# Autodesk Inventor assembly: Swerve-Drivetrain-2
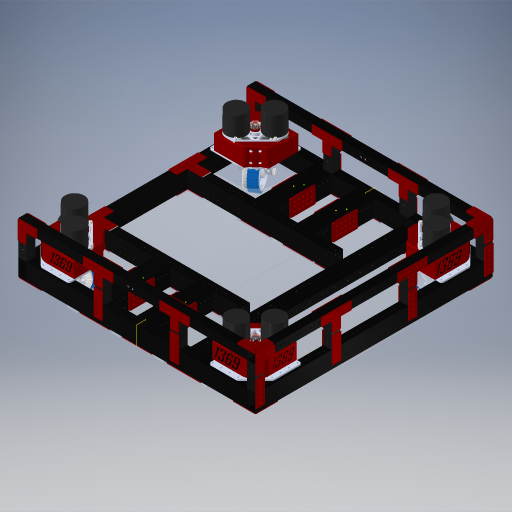
[picture p0: Inventor's stored thumbnail of the model, 512x512]
Saved by Autodesk Inventor 2024.2 (Build 282272000, 272)
## iProperties
Created: 2024-01-06
Part Number: Swerve-Drivetrain-2
Document SubType Name: Assembly
Designer: rohan
Author: rohan
## Documents named in this file (18)
- C:\Users\rohan\OneDrive - Hillsborough County Public Schools\Robotics\FIRST-Robotics-Competition\Crescendo\Minotaur-Crescendo-Robot\Swerve-Drivetrain.iam
- C:\Users\rohan\OneDrive - Hillsborough County Public Schools\Robotics\FIRST-Robotics-Competition\Crescendo\Minotaur-Crescendo-Robot\Motion\SDS-Swerve-Modules\MK3-Swerve-Module-Neos.iam
- C:\Users\rohan\OneDrive - Hillsborough County Public Schools\Robotics\FIRST-Robotics-Competition\Crescendo\Minotaur-Crescendo-Robot\Structure\Aluminum-Extrusions\2024-100-002-Front-Back-Extrusions.ipt
- C:\Users\rohan\OneDrive - Hillsborough County Public Schools\Robotics\FIRST-Robotics-Competition\Crescendo\Minotaur-Crescendo-Robot\Structure\Aluminum-Extrusions\2024-100-001-Left-Right-Extrusions.ipt
- C:\Users\rohan\OneDrive - Hillsborough County Public Schools\Robotics\FIRST-Robotics-Competition\Crescendo\Minotaur-Crescendo-Robot\Structure\Aluminum-Extrusions\2024-100-003-Middle-Extrusions.ipt
- C:\Users\rohan\OneDrive - Hillsborough County Public Schools\Robotics\FIRST-Robotics-Competition\Crescendo\Minotaur-Crescendo-Robot\Structure\Gussets\THRIFYBOT-L-Gusset.ipt
- C:\Users\rohan\OneDrive - Hillsborough County Public Schools\Robotics\FIRST-Robotics-Competition\Crescendo\Minotaur-Crescendo-Robot\Structure\Bumpers.ipt
- C:\Users\rohan\OneDrive - Hillsborough County Public Schools\Robotics\FIRST-Robotics-Competition\Crescendo\Minotaur-Crescendo-Robot\Structure\Aluminum-Extrusions\2024-100-007-Front-B-Tubing-Mount.ipt
- C:\Users\rohan\OneDrive - Hillsborough County Public Schools\Robotics\FIRST-Robotics-Competition\Crescendo\Minotaur-Crescendo-Robot\Structure\Gussets\THRIFYBOT-T-Gusset.ipt
- C:\Users\rohan\OneDrive - Hillsborough County Public Schools\Robotics\FIRST-Robotics-Competition\Crescendo\Minotaur-Crescendo-Robot\Structure\Gussets\Custom-Underside-T-Gusset.ipt
- C:\Users\rohan\OneDrive - Hillsborough County Public Schools\Robotics\FIRST-Robotics-Competition\Crescendo\Minotaur-Crescendo-Robot\Structure\Gussets\Custom-Underside-L-Gusset.ipt
- C:\Users\rohan\OneDrive - Hillsborough County Public Schools\Robotics\FIRST-Robotics-Competition\Crescendo\Minotaur-Crescendo-Robot\Structure\Aluminum-Extrusions\Superstructure-Mount.iam
- C:\Users\rohan\OneDrive - Hillsborough County Public Schools\Robotics\FIRST-Robotics-Competition\Crescendo\Minotaur-Crescendo-Robot\Structure\Gussets\3x5-Grid-Gusset.ipt
- C:\Users\rohan\OneDrive - Hillsborough County Public Schools\Robotics\FIRST-Robotics-Competition\Crescendo\Minotaur-Crescendo-Robot\Structure\Aluminum-Extrusions\2024-100-005-Climber-Mount.ipt
- C:\Users\rohan\OneDrive - Hillsborough County Public Schools\Robotics\FIRST-Robotics-Competition\Crescendo\Minotaur-Crescendo-Robot\Structure\Aluminum-Extrusions\2024-100-010-Climber-Support.ipt
- C:\Users\rohan\OneDrive - Hillsborough County Public Schools\Robotics\FIRST-Robotics-Competition\Crescendo\Minotaur-Crescendo-Robot\Structure\Gussets\1x5-Grid-Gusset.ipt
- C:\Users\rohan\OneDrive - Hillsborough County Public Schools\Robotics\FIRST-Robotics-Competition\Crescendo\Minotaur-Crescendo-Robot\Structure\Aluminum-Plates\2024-100-006-Electrical-Plate-Bottom.ipt
- C:\Users\rohan\OneDrive - Hillsborough County Public Schools\Robotics\FIRST-Robotics-Competition\Crescendo\Minotaur-Crescendo-Robot\Structure\Aluminum-Plates\2024-100-006-Electrical-Plate-Front.ipt
## Components (61 placed, 17 different names)
1. MK3-Swerve-Module-Neos:1 [sub-assembly] — Mate:75, Mate:80, Mate:81
2. MK3-Swerve-Module-Neos:2 [sub-assembly] — Mate:74, Mate:82, Mate:83
3. MK3-Swerve-Module-Neos:3 [sub-assembly] — Mate:73, Mate:76, Mate:77
4. MK3-Swerve-Module-Neos:4 [sub-assembly] — Mate:72, Mate:78, Mate:79
5. 2024-100-001-Left-Right-Extrusions:1 — Mate:69, Flush:1, Flush:2, Mate:70, Flush:3, Flush:4, Mate:73, Mate:76, Mate:82, Flush:12, Flush:14, Flush:45, Mate:111, Flush:53, Flush:54, Mate:147, Mate:148, Mate:149, Flush:106, Flush:107, Insert:14, Insert:15, Mate:165, Mate:166
6. 2024-100-001-Left-Right-Extrusions:2 — Mate:71, Flush:5, Flush:6, Mate:79, Mate:81, Flush:10, Flush:16, Mate:99, Mate:106, Flush:51, Flush:88, Flush:91, Mate:157, Mate:158, Flush:109, Flush:111
7. 2024-100-002-Front-Back-Extrusions:1 — Mate:70, Flush:3, Flush:4, Mate:72, Mate:77, Mate:78, Mate:88, Mate:89, Flush:13, Flush:15, Flush:33, Mate:112, Mate:159, Mate:160, Mate:161, Mate:162, Mate:163, Mate:164, Flush:110
8. 2024-100-002-Front-Back-Extrusions:2 — Mate:69, Flush:1, Flush:2, Mate:71, Flush:5, Flush:6, Mate:74, Mate:75, Mate:80, Mate:83, Mate:86, Mate:87, Flush:9, Flush:11, Mate:98, Mate:101, Flush:38, Flush:40, Insert:1, Flush:43, Mate:105, Insert:2, Flush:55, Mate:123, Mate:167, Flush:108
9. THRIFYBOT-L-Gusset:1 — Mate:89, Flush:13, Flush:14
10. THRIFYBOT-L-Gusset:2 — Mate:88, Flush:15, Flush:16
11. THRIFYBOT-L-Gusset:3 — Mate:87, Flush:11, Flush:12
12. THRIFYBOT-L-Gusset:4 — Mate:86, Flush:9, Flush:10
13. Bumpers:1 — Mate:98, Mate:99, Flush:33
14. 2024-100-007-Front-B-Tubing-Mount:1 — Mate:100, Flush:34, Mate:101, Flush:35, Flush:39, Mate:103, Flush:40, Mate:107, Flush:48, Insert:3, Mate:121, Flush:70, Mate:136, Flush:87, Flush:89, Mate:140, Flush:90, Insert:20
15. 2024-100-007-Front-B-Tubing-Mount:2 — Mate:100, Flush:34, Flush:35, Flush:44, Flush:47, Insert:4, Flush:102, Flush:103, Flush:104, Flush:105, Insert:16, Insert:17
16. THRIFYBOT-T-Gusset:1 — Flush:36, Mate:102, Flush:37, Mate:103
17. THRIFYBOT-T-Gusset:2 — Flush:36, Mate:102, Flush:37, Flush:38, Flush:39, Insert:1
18. THRIFYBOT-T-Gusset:3 — Mate:105
19. THRIFYBOT-T-Gusset:4 — Flush:43, Flush:44, Insert:2
20. 2024-100-003-Middle-Extrusions:1 — Flush:45, Mate:106, Mate:107, Mate:108, Mate:109, Flush:46, Flush:49, Mate:110, Flush:50, Flush:52, Mate:168
21. Custom-Underside-T-Gusset:1 — Mate:108, Flush:48, Flush:49, Insert:3
22. Custom-Underside-T-Gusset:2 — Mate:109, Flush:46, Flush:47, Insert:4
23. Custom-Underside-L-Gusset:4 — Mate:111, Flush:52, Flush:53
24. Custom-Underside-L-Gusset:5 — Mate:110, Flush:50, Flush:51
25. Superstructure-Mount:1 [sub-assembly] — Mate:112, Flush:54, Flush:55, Insert:21, Insert:22, Insert:23, Insert:24, Insert:25, Insert:26, Insert:27, Insert:28, Insert:29, Insert:30, Insert:31, Insert:32, Insert:33, Insert:34, Insert:35, Insert:36, Insert:37, Insert:38, Insert:39, Insert:40
26. 3x5-Grid-Gusset:3
27. 3x5-Grid-Gusset:4
28. 2024-100-005-Climber-Mount:2 — Flush:70, Mate:123
29. 2024-100-010-Climber-Support:2 — Mate:121, Mate:137, Mate:138, Insert:10, Insert:11
30. 3x5-Grid-Gusset:5
31. 3x5-Grid-Gusset:6
32. 2024-100-005-Climber-Mount:3 — Mate:136, Flush:87
33. 2024-100-010-Climber-Support:3 — Mate:139, Insert:8, Insert:9
34. THRIFYBOT-T-Gusset:5 — Mate:139, Flush:91, Insert:8
35. THRIFYBOT-T-Gusset:6 — Flush:89, Mate:138, Insert:11
36. THRIFYBOT-T-Gusset:7 — Mate:140, Flush:90, Insert:9, Insert:20
37. THRIFYBOT-T-Gusset:8 — Mate:137, Flush:88, Insert:10
38. 3x5-Grid-Gusset:7
39. 3x5-Grid-Gusset:8
40. 2024-100-005-Climber-Mount:4 — Mate:147, Flush:103
41. 2024-100-010-Climber-Support:4 — Mate:150, Mate:152, Insert:18
42. 3x5-Grid-Gusset:9
43. 3x5-Grid-Gusset:10
44. 2024-100-005-Climber-Mount:5 — Flush:102
45. 2024-100-010-Climber-Support:5 — Mate:148, Mate:151, Insert:19
46. THRIFYBOT-T-Gusset:9 — Mate:149, Flush:106, Insert:15, Insert:19
47. THRIFYBOT-T-Gusset:10 — Mate:151, Flush:105, Insert:16
48. THRIFYBOT-T-Gusset:11 — Mate:150, Flush:107, Insert:14, Insert:18
49. THRIFYBOT-T-Gusset:12 — Mate:152, Flush:104, Insert:17
50. 1x5-Grid-Gusset:1 — Mate:157, Insert:21, Insert:22
51. 1x5-Grid-Gusset:2 — Mate:158, Insert:23, Insert:24
52. 1x5-Grid-Gusset:3 — Mate:159, Insert:27, Insert:28
53. 1x5-Grid-Gusset:4 — Mate:160, Insert:25, Insert:26
54. 1x5-Grid-Gusset:5 — Mate:161, Insert:31, Insert:32
55. 1x5-Grid-Gusset:6 — Mate:162, Insert:29, Insert:30
56. 1x5-Grid-Gusset:7 — Mate:163, Insert:33, Insert:34
57. 1x5-Grid-Gusset:8 — Mate:164, Insert:35, Insert:36
58. 1x5-Grid-Gusset:10 — Mate:166, Insert:37, Insert:38
59. 1x5-Grid-Gusset:11 — Mate:165, Insert:39, Insert:40
60. 2024-100-006-Electrical-Plate-Bottom:1 — Mate:168, Flush:110, Flush:111
61. 2024-100-006-Electrical-Plate-Front:1 — Mate:167, Flush:108, Flush:109
## Relationships (183: Flush 73, Mate 71, Insert 39)
- Mate:69: 2024-100-001-Left-Right-Extrusions:1 ↔ 2024-100-002-Front-Back-Extrusions:2
- Flush:1: 2024-100-001-Left-Right-Extrusions:1 ↔ 2024-100-002-Front-Back-Extrusions:2
- Flush:2: 2024-100-001-Left-Right-Extrusions:1 ↔ 2024-100-002-Front-Back-Extrusions:2
- Mate:70: 2024-100-001-Left-Right-Extrusions:1 ↔ 2024-100-002-Front-Back-Extrusions:1
- Flush:3: 2024-100-001-Left-Right-Extrusions:1 ↔ 2024-100-002-Front-Back-Extrusions:1
- Flush:4: 2024-100-001-Left-Right-Extrusions:1 ↔ 2024-100-002-Front-Back-Extrusions:1
- Mate:71: 2024-100-001-Left-Right-Extrusions:2 ↔ 2024-100-002-Front-Back-Extrusions:2
- Flush:5: 2024-100-001-Left-Right-Extrusions:2 ↔ 2024-100-002-Front-Back-Extrusions:2
- Flush:6: 2024-100-001-Left-Right-Extrusions:2 ↔ 2024-100-002-Front-Back-Extrusions:2
- Mate:72: MK3-Swerve-Module-Neos:4 ↔ 2024-100-002-Front-Back-Extrusions:1
- Mate:73: MK3-Swerve-Module-Neos:3 ↔ 2024-100-001-Left-Right-Extrusions:1
- Mate:74: MK3-Swerve-Module-Neos:2 ↔ 2024-100-002-Front-Back-Extrusions:2
- Mate:75: MK3-Swerve-Module-Neos:1 ↔ 2024-100-002-Front-Back-Extrusions:2
- Mate:76: MK3-Swerve-Module-Neos:3 ↔ 2024-100-001-Left-Right-Extrusions:1
- Mate:77: MK3-Swerve-Module-Neos:3 ↔ 2024-100-002-Front-Back-Extrusions:1
- Mate:78: MK3-Swerve-Module-Neos:4 ↔ 2024-100-002-Front-Back-Extrusions:1
- Mate:79: MK3-Swerve-Module-Neos:4 ↔ 2024-100-001-Left-Right-Extrusions:2
- Mate:80: MK3-Swerve-Module-Neos:1 ↔ 2024-100-002-Front-Back-Extrusions:2
- Mate:81: MK3-Swerve-Module-Neos:1 ↔ 2024-100-001-Left-Right-Extrusions:2
- Mate:82: MK3-Swerve-Module-Neos:2 ↔ 2024-100-001-Left-Right-Extrusions:1
- Mate:83: MK3-Swerve-Module-Neos:2 ↔ 2024-100-002-Front-Back-Extrusions:2
- Mate:86: 2024-100-002-Front-Back-Extrusions:2 ↔ THRIFYBOT-L-Gusset:4
- Mate:87: 2024-100-002-Front-Back-Extrusions:2 ↔ THRIFYBOT-L-Gusset:3
- Mate:88: 2024-100-002-Front-Back-Extrusions:1 ↔ THRIFYBOT-L-Gusset:2
- Mate:89: 2024-100-002-Front-Back-Extrusions:1 ↔ THRIFYBOT-L-Gusset:1
- Flush:9: 2024-100-002-Front-Back-Extrusions:2 ↔ THRIFYBOT-L-Gusset:4
- Flush:10: 2024-100-001-Left-Right-Extrusions:2 ↔ THRIFYBOT-L-Gusset:4
- Flush:11: 2024-100-002-Front-Back-Extrusions:2 ↔ THRIFYBOT-L-Gusset:3
- Flush:12: 2024-100-001-Left-Right-Extrusions:1 ↔ THRIFYBOT-L-Gusset:3
- Flush:13: 2024-100-002-Front-Back-Extrusions:1 ↔ THRIFYBOT-L-Gusset:1
- Flush:14: 2024-100-001-Left-Right-Extrusions:1 ↔ THRIFYBOT-L-Gusset:1
- Flush:15: 2024-100-002-Front-Back-Extrusions:1 ↔ THRIFYBOT-L-Gusset:2
- Flush:16: 2024-100-001-Left-Right-Extrusions:2 ↔ THRIFYBOT-L-Gusset:2
- Mate:98: 2024-100-002-Front-Back-Extrusions:2 ↔ Bumpers:1
- Mate:99: 2024-100-001-Left-Right-Extrusions:2 ↔ Bumpers:1
- Flush:33 (63.5 mm): 2024-100-002-Front-Back-Extrusions:1 ↔ Bumpers:1
- Mate:100 (254 mm): 2024-100-007-Front-B-Tubing-Mount:1 ↔ 2024-100-007-Front-B-Tubing-Mount:2
- Flush:34: 2024-100-007-Front-B-Tubing-Mount:1 ↔ 2024-100-007-Front-B-Tubing-Mount:2
- Mate:101: 2024-100-002-Front-Back-Extrusions:2 ↔ 2024-100-007-Front-B-Tubing-Mount:1
- Flush:35: 2024-100-007-Front-B-Tubing-Mount:1 ↔ 2024-100-007-Front-B-Tubing-Mount:2
- Flush:36: THRIFYBOT-T-Gusset:1 ↔ THRIFYBOT-T-Gusset:2
- Mate:102 (50.8 mm): THRIFYBOT-T-Gusset:1 ↔ THRIFYBOT-T-Gusset:2
- Flush:37: THRIFYBOT-T-Gusset:1 ↔ THRIFYBOT-T-Gusset:2
- Flush:38: 2024-100-002-Front-Back-Extrusions:2 ↔ THRIFYBOT-T-Gusset:2
- Flush:39: 2024-100-007-Front-B-Tubing-Mount:1 ↔ THRIFYBOT-T-Gusset:2
- Mate:103: 2024-100-007-Front-B-Tubing-Mount:1 ↔ THRIFYBOT-T-Gusset:1
- Flush:40: 2024-100-002-Front-Back-Extrusions:2 ↔ 2024-100-007-Front-B-Tubing-Mount:1
- Insert:1: 2024-100-002-Front-Back-Extrusions:2 ↔ THRIFYBOT-T-Gusset:2
- [Flush]: THRIFYBOT-T-Gusset:3 ↔ THRIFYBOT-T-Gusset:4
- [Mate] (50.8 mm): THRIFYBOT-T-Gusset:3 ↔ THRIFYBOT-T-Gusset:4
- [Flush]: THRIFYBOT-T-Gusset:3 ↔ THRIFYBOT-T-Gusset:4
- Flush:43: 2024-100-002-Front-Back-Extrusions:2 ↔ THRIFYBOT-T-Gusset:4
- Flush:44: 2024-100-007-Front-B-Tubing-Mount:2 ↔ THRIFYBOT-T-Gusset:4
- Mate:105: 2024-100-002-Front-Back-Extrusions:2 ↔ THRIFYBOT-T-Gusset:3
- Insert:2: 2024-100-002-Front-Back-Extrusions:2 ↔ THRIFYBOT-T-Gusset:4
- Flush:45: 2024-100-001-Left-Right-Extrusions:1 ↔ 2024-100-003-Middle-Extrusions:1
- Mate:106: 2024-100-001-Left-Right-Extrusions:2 ↔ 2024-100-003-Middle-Extrusions:1
- Mate:107: 2024-100-007-Front-B-Tubing-Mount:1 ↔ 2024-100-003-Middle-Extrusions:1
- Mate:108: 2024-100-003-Middle-Extrusions:1 ↔ Custom-Underside-T-Gusset:1
- Mate:109: 2024-100-003-Middle-Extrusions:1 ↔ Custom-Underside-T-Gusset:2
- Flush:46: 2024-100-003-Middle-Extrusions:1 ↔ Custom-Underside-T-Gusset:2
- Flush:47: 2024-100-007-Front-B-Tubing-Mount:2 ↔ Custom-Underside-T-Gusset:2
- Flush:48: 2024-100-007-Front-B-Tubing-Mount:1 ↔ Custom-Underside-T-Gusset:1
- Flush:49: 2024-100-003-Middle-Extrusions:1 ↔ Custom-Underside-T-Gusset:1
- Insert:3: 2024-100-007-Front-B-Tubing-Mount:1 ↔ Custom-Underside-T-Gusset:1
- Insert:4: 2024-100-007-Front-B-Tubing-Mount:2 ↔ Custom-Underside-T-Gusset:2
- Mate:110: 2024-100-003-Middle-Extrusions:1 ↔ Custom-Underside-L-Gusset:5
- Flush:50: 2024-100-003-Middle-Extrusions:1 ↔ Custom-Underside-L-Gusset:5
- Flush:51: 2024-100-001-Left-Right-Extrusions:2 ↔ Custom-Underside-L-Gusset:5
- Mate:111: 2024-100-001-Left-Right-Extrusions:1 ↔ Custom-Underside-L-Gusset:4
- Flush:52: 2024-100-003-Middle-Extrusions:1 ↔ Custom-Underside-L-Gusset:4
- Flush:53: 2024-100-001-Left-Right-Extrusions:1 ↔ Custom-Underside-L-Gusset:4
- Mate:112: 2024-100-002-Front-Back-Extrusions:1 ↔ Superstructure-Mount:1
- Flush:54: 2024-100-001-Left-Right-Extrusions:1 ↔ Superstructure-Mount:1
- Flush:55: 2024-100-002-Front-Back-Extrusions:2 ↔ Superstructure-Mount:1
- [Flush]: 3x5-Grid-Gusset:3 ↔ 3x5-Grid-Gusset:4
- [Flush]: 3x5-Grid-Gusset:3 ↔ 3x5-Grid-Gusset:4
- [Mate] (50.8 mm): 3x5-Grid-Gusset:3 ↔ 3x5-Grid-Gusset:4
- [Flush]: 2024-100-005-Climber-Mount:2 ↔ 2024-100-010-Climber-Support:2
- [Flush]: 2024-100-005-Climber-Mount:2 ↔ 2024-100-010-Climber-Support:2
- [Mate]: 2024-100-005-Climber-Mount:2 ↔ 2024-100-010-Climber-Support:2
- [Flush]: 3x5-Grid-Gusset:4 ↔ 2024-100-005-Climber-Mount:2
- [Mate]: 3x5-Grid-Gusset:3 ↔ 2024-100-005-Climber-Mount:2
- [Insert]: 3x5-Grid-Gusset:4 ↔ 2024-100-005-Climber-Mount:2
- Mate:121: 2024-100-007-Front-B-Tubing-Mount:1 ↔ 2024-100-010-Climber-Support:2
- Flush:70: 2024-100-007-Front-B-Tubing-Mount:1 ↔ 2024-100-005-Climber-Mount:2
- Mate:123 (304.8 mm): 2024-100-002-Front-Back-Extrusions:2 ↔ 2024-100-005-Climber-Mount:2
- [Flush]: 3x5-Grid-Gusset:5 ↔ 3x5-Grid-Gusset:6
- [Flush]: 3x5-Grid-Gusset:5 ↔ 3x5-Grid-Gusset:6
- [Mate] (50.8 mm): 3x5-Grid-Gusset:5 ↔ 3x5-Grid-Gusset:6
- [Flush]: 2024-100-005-Climber-Mount:3 ↔ 2024-100-010-Climber-Support:3
- [Flush]: 2024-100-005-Climber-Mount:3 ↔ 2024-100-010-Climber-Support:3
- [Mate]: 2024-100-005-Climber-Mount:3 ↔ 2024-100-010-Climber-Support:3
- [Flush]: 3x5-Grid-Gusset:6 ↔ 2024-100-005-Climber-Mount:3
- [Mate]: 3x5-Grid-Gusset:5 ↔ 2024-100-005-Climber-Mount:3
- [Insert]: 3x5-Grid-Gusset:6 ↔ 2024-100-005-Climber-Mount:3
- Mate:136: 2024-100-007-Front-B-Tubing-Mount:1 ↔ 2024-100-005-Climber-Mount:3
- Flush:87: 2024-100-007-Front-B-Tubing-Mount:1 ↔ 2024-100-005-Climber-Mount:3
- Mate:137: 2024-100-010-Climber-Support:2 ↔ THRIFYBOT-T-Gusset:8
- Flush:88: 2024-100-001-Left-Right-Extrusions:2 ↔ THRIFYBOT-T-Gusset:8
- Flush:89: 2024-100-007-Front-B-Tubing-Mount:1 ↔ THRIFYBOT-T-Gusset:6
- Mate:138: 2024-100-010-Climber-Support:2 ↔ THRIFYBOT-T-Gusset:6
- Mate:139: 2024-100-010-Climber-Support:3 ↔ THRIFYBOT-T-Gusset:5
- Mate:140: 2024-100-007-Front-B-Tubing-Mount:1 ↔ THRIFYBOT-T-Gusset:7
- Flush:90: 2024-100-007-Front-B-Tubing-Mount:1 ↔ THRIFYBOT-T-Gusset:7
- Flush:91: 2024-100-001-Left-Right-Extrusions:2 ↔ THRIFYBOT-T-Gusset:5
- Insert:8: 2024-100-010-Climber-Support:3 ↔ THRIFYBOT-T-Gusset:5
- Insert:9: 2024-100-010-Climber-Support:3 ↔ THRIFYBOT-T-Gusset:7
- Insert:10: 2024-100-010-Climber-Support:2 ↔ THRIFYBOT-T-Gusset:8
- Insert:11: 2024-100-010-Climber-Support:2 ↔ THRIFYBOT-T-Gusset:6
- [Flush]: 3x5-Grid-Gusset:7 ↔ 3x5-Grid-Gusset:8
- [Flush]: 3x5-Grid-Gusset:7 ↔ 3x5-Grid-Gusset:8
- [Mate] (50.8 mm): 3x5-Grid-Gusset:7 ↔ 3x5-Grid-Gusset:8
- [Flush]: 2024-100-005-Climber-Mount:4 ↔ 2024-100-010-Climber-Support:4
- [Flush]: 2024-100-005-Climber-Mount:4 ↔ 2024-100-010-Climber-Support:4
- [Mate]: 2024-100-005-Climber-Mount:4 ↔ 2024-100-010-Climber-Support:4
- [Flush]: 3x5-Grid-Gusset:8 ↔ 2024-100-005-Climber-Mount:4
- [Mate]: 3x5-Grid-Gusset:7 ↔ 2024-100-005-Climber-Mount:4
- [Insert]: 3x5-Grid-Gusset:8 ↔ 2024-100-005-Climber-Mount:4
- [Flush]: 3x5-Grid-Gusset:9 ↔ 3x5-Grid-Gusset:10
- [Flush]: 3x5-Grid-Gusset:9 ↔ 3x5-Grid-Gusset:10
- [Mate] (50.8 mm): 3x5-Grid-Gusset:9 ↔ 3x5-Grid-Gusset:10
- [Flush]: 2024-100-005-Climber-Mount:5 ↔ 2024-100-010-Climber-Support:5
- [Flush]: 2024-100-005-Climber-Mount:5 ↔ 2024-100-010-Climber-Support:5
- [Mate]: 2024-100-005-Climber-Mount:5 ↔ 2024-100-010-Climber-Support:5
- [Flush]: 3x5-Grid-Gusset:10 ↔ 2024-100-005-Climber-Mount:5
- [Mate]: 3x5-Grid-Gusset:9 ↔ 2024-100-005-Climber-Mount:5
- [Insert]: 3x5-Grid-Gusset:10 ↔ 2024-100-005-Climber-Mount:5
- Mate:147: 2024-100-001-Left-Right-Extrusions:1 ↔ 2024-100-005-Climber-Mount:4
- Mate:148: 2024-100-001-Left-Right-Extrusions:1 ↔ 2024-100-010-Climber-Support:5
- Flush:102: 2024-100-007-Front-B-Tubing-Mount:2 ↔ 2024-100-005-Climber-Mount:5
- Flush:103: 2024-100-007-Front-B-Tubing-Mount:2 ↔ 2024-100-005-Climber-Mount:4
- Mate:149: 2024-100-001-Left-Right-Extrusions:1 ↔ THRIFYBOT-T-Gusset:9
- Mate:150: 2024-100-010-Climber-Support:4 ↔ THRIFYBOT-T-Gusset:11
- Mate:151: 2024-100-010-Climber-Support:5 ↔ THRIFYBOT-T-Gusset:10
- Mate:152: 2024-100-010-Climber-Support:4 ↔ THRIFYBOT-T-Gusset:12
- Flush:104: 2024-100-007-Front-B-Tubing-Mount:2 ↔ THRIFYBOT-T-Gusset:12
- Flush:105: 2024-100-007-Front-B-Tubing-Mount:2 ↔ THRIFYBOT-T-Gusset:10
- Flush:106: 2024-100-001-Left-Right-Extrusions:1 ↔ THRIFYBOT-T-Gusset:9
- Flush:107: 2024-100-001-Left-Right-Extrusions:1 ↔ THRIFYBOT-T-Gusset:11
- Insert:14: 2024-100-001-Left-Right-Extrusions:1 ↔ THRIFYBOT-T-Gusset:11
- Insert:15: 2024-100-001-Left-Right-Extrusions:1 ↔ THRIFYBOT-T-Gusset:9
- Insert:16: 2024-100-007-Front-B-Tubing-Mount:2 ↔ THRIFYBOT-T-Gusset:10
- Insert:17: 2024-100-007-Front-B-Tubing-Mount:2 ↔ THRIFYBOT-T-Gusset:12
- Insert:18: 2024-100-010-Climber-Support:4 ↔ THRIFYBOT-T-Gusset:11
- Insert:19: 2024-100-010-Climber-Support:5 ↔ THRIFYBOT-T-Gusset:9
- Insert:20: 2024-100-007-Front-B-Tubing-Mount:1 ↔ THRIFYBOT-T-Gusset:7
- Mate:157: 2024-100-001-Left-Right-Extrusions:2 ↔ 1x5-Grid-Gusset:1
- Insert:21: Superstructure-Mount:1 ↔ 1x5-Grid-Gusset:1
- Insert:22: Superstructure-Mount:1 ↔ 1x5-Grid-Gusset:1
- Mate:158: 2024-100-001-Left-Right-Extrusions:2 ↔ 1x5-Grid-Gusset:2
- Insert:23: Superstructure-Mount:1 ↔ 1x5-Grid-Gusset:2
- Insert:24: Superstructure-Mount:1 ↔ 1x5-Grid-Gusset:2
- Mate:159: 2024-100-002-Front-Back-Extrusions:1 ↔ 1x5-Grid-Gusset:3
- Mate:160: 2024-100-002-Front-Back-Extrusions:1 ↔ 1x5-Grid-Gusset:4
- Insert:25: Superstructure-Mount:1 ↔ 1x5-Grid-Gusset:4
- Insert:26: Superstructure-Mount:1 ↔ 1x5-Grid-Gusset:4
- Insert:27: Superstructure-Mount:1 ↔ 1x5-Grid-Gusset:3
- Insert:28: Superstructure-Mount:1 ↔ 1x5-Grid-Gusset:3
- Mate:161: 2024-100-002-Front-Back-Extrusions:1 ↔ 1x5-Grid-Gusset:5
- Mate:162: 2024-100-002-Front-Back-Extrusions:1 ↔ 1x5-Grid-Gusset:6
- Insert:29: Superstructure-Mount:1 ↔ 1x5-Grid-Gusset:6
- Insert:30: Superstructure-Mount:1 ↔ 1x5-Grid-Gusset:6
- Insert:31: Superstructure-Mount:1 ↔ 1x5-Grid-Gusset:5
- Insert:32: Superstructure-Mount:1 ↔ 1x5-Grid-Gusset:5
- Mate:163: 2024-100-002-Front-Back-Extrusions:1 ↔ 1x5-Grid-Gusset:7
- Insert:33: Superstructure-Mount:1 ↔ 1x5-Grid-Gusset:7
- Insert:34: Superstructure-Mount:1 ↔ 1x5-Grid-Gusset:7
- Mate:164: 2024-100-002-Front-Back-Extrusions:1 ↔ 1x5-Grid-Gusset:8
- Insert:35: Superstructure-Mount:1 ↔ 1x5-Grid-Gusset:8
- Insert:36: Superstructure-Mount:1 ↔ 1x5-Grid-Gusset:8
- Mate:165: 2024-100-001-Left-Right-Extrusions:1 ↔ 1x5-Grid-Gusset:11
- Mate:166: 2024-100-001-Left-Right-Extrusions:1 ↔ 1x5-Grid-Gusset:10
- Insert:37: Superstructure-Mount:1 ↔ 1x5-Grid-Gusset:10
- Insert:38: Superstructure-Mount:1 ↔ 1x5-Grid-Gusset:10
- Insert:39: Superstructure-Mount:1 ↔ 1x5-Grid-Gusset:11
- Insert:40: Superstructure-Mount:1 ↔ 1x5-Grid-Gusset:11
- Mate:167: 2024-100-002-Front-Back-Extrusions:2 ↔ 2024-100-006-Electrical-Plate-Front:1
- Flush:108: 2024-100-002-Front-Back-Extrusions:2 ↔ 2024-100-006-Electrical-Plate-Front:1
- Flush:109: 2024-100-001-Left-Right-Extrusions:2 ↔ 2024-100-006-Electrical-Plate-Front:1
- Mate:168: 2024-100-003-Middle-Extrusions:1 ↔ 2024-100-006-Electrical-Plate-Bottom:1
- Flush:110: 2024-100-002-Front-Back-Extrusions:1 ↔ 2024-100-006-Electrical-Plate-Bottom:1
- Flush:111: 2024-100-001-Left-Right-Extrusions:2 ↔ 2024-100-006-Electrical-Plate-Bottom:1
## Named parameters: d320_d312 = 0 mm, d321_d313 = 50.8 mm, d322_d314 = 0 mm, d377_d362 = 0 mm, d378_d363 = 0 mm, d379_d364 = 50.8 mm, d380_d368 = 0 mm, d381_d369 = 0 mm, d382_d370 = 0 mm, d383_d374 = 0 mm, d384_d375 = 0 mm, d385_d376 = 0 mm, d423_d377_d362 = 0 mm, d424_d378_d363 = 0 mm, d425_d379_d364 = 50.8 mm, d426_d380_d368 = 0 mm, d427_d381_d369 = 0 mm, d428_d382_d370 = 0 mm, d429_d383_d374 = 0 mm, d430_d384_d375 = 0 mm, d431_d385_d376 = 0 mm, d449_d423_d377_d362 = 0 mm, d450_d424_d378_d363 = 0 mm, d451_d425_d379_d364 = 50.8 mm, d452_d426_d380_d368 = 0 mm, d453_d427_d381_d369 = 0 mm, d454_d428_d382_d370 = 0 mm, d455_d429_d383_d374 = 0 mm, d456_d430_d384_d375 = 0 mm, d457_d431_d385_d376 = 0 mm, d458_d423_d377_d362 = 0 mm, d459_d424_d378_d363 = 0 mm, d460_d425_d379_d364 = 50.8 mm, d461_d426_d380_d368 = 0 mm, d462_d427_d381_d369 = 0 mm, d463_d428_d382_d370 = 0 mm, d464_d429_d383_d374 = 0 mm, d465_d430_d384_d375 = 0 mm, d466_d431_d385_d376 = 0 mm
